# Autodesk Inventor assembly: ShootingMech_Detailed
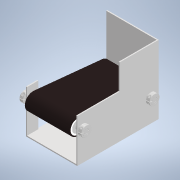
[picture p0: Inventor's stored thumbnail of the model, 180x180]
Saved by Autodesk Inventor 2020 (Build 240168000, 168)
## iProperties
Created: 2022-01-26
Part Number: ShootingMech_Detailed
Document SubType Name: Assembly
Designer: danie
Author: danie
## Documents named in this file (4)
- C:\Users\danie\Documents\Capstone\Solidworks\ShootingMech_Detailed.iam
- C:\Users\danie\Documents\Capstone\Solidworks\Shooting_Case.ipt
- C:\Users\danie\Documents\Capstone\Solidworks\Shooting_BeltandBearings.iam
- C:\Users\danie\Documents\Capstone\Solidworks\6435K14_Clamping Shaft Collar.ipt
## Components (5 placed, 3 different names)
1. Shooting_Case:1
2. Shooting_BeltandBearings:1 [sub-assembly] — Rotational:1, Rigid:1, Rigid:2
3. 6435K14_Clamping Shaft Collar:1 — Rotational:1
4. 6435K14_Clamping Shaft Collar:2 — Rigid:2
5. 6435K14_Clamping Shaft Collar:3 — Rigid:1
## Relationships (3: WeldJoint 2, RevoluteJoint 1)
- Rotational:1 [RevoluteJoint]: Shooting_BeltandBearings:1 ↔ 6435K14_Clamping Shaft Collar:1
- Rigid:1 [WeldJoint]: Shooting_BeltandBearings:1 ↔ 6435K14_Clamping Shaft Collar:3
- Rigid:2 [WeldJoint]: Shooting_BeltandBearings:1 ↔ 6435K14_Clamping Shaft Collar:2
